# Autodesk Inventor assembly: sholder
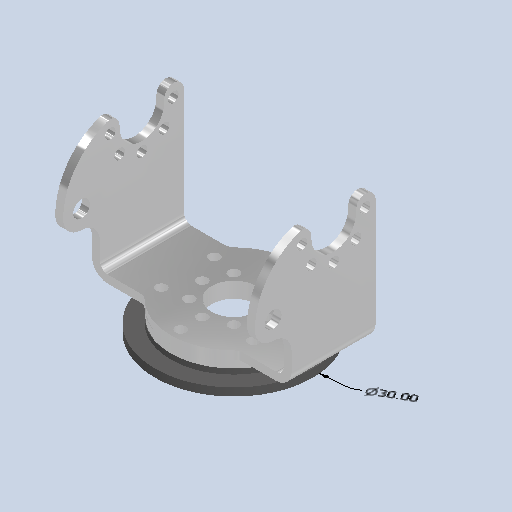
[picture p0: Inventor's stored thumbnail of the model, 512x512]
Saved by Autodesk Inventor 2024.1 (Build 281209000, 209)
## iProperties
Created: 2024-10-10
Part Number: sholder
Document SubType Name: Assembly
Designer: hibik
Author: hibik
## Documents named in this file (4)
- C:\Users\hibik\Documents\Robomech\HR\Eglantyne\hard\upper_body\sholder.iam
- C:\Users\hibik\Documents\Robomech\HR\Eglantyne\hard\upper_body\sholder.ipt
- C:\Users\hibik\Documents\Robomech\HR\Eglantyne\hard\common_parts\joint_setter_c.ipt
- C:\Users\hibik\Documents\Robomech\HR\Eglantyne\hard\common_parts\joint_setter_s.ipt
## Components (3 placed, 3 different names)
1. sholder:1 — 挿入:1, 挿入:2
2. joint_setter_c:1 — 挿入:3, 挿入:4
3. joint_setter_s:1 — 挿入:1, 挿入:2, 挿入:3, 挿入:4
## Relationships (4: Insert 4)
- 挿入:1 [Insert]: sholder:1 ↔ joint_setter_s:1
- 挿入:2 [Insert]: sholder:1 ↔ joint_setter_s:1
- 挿入:3 [Insert]: joint_setter_c:1 ↔ joint_setter_s:1
- 挿入:4 [Insert]: joint_setter_c:1 ↔ joint_setter_s:1
